# Autodesk Inventor assembly: BatteryPack
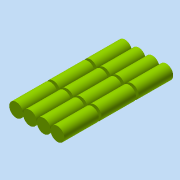
[picture p0: Inventor's stored thumbnail of the model, 180x180]
Saved by Autodesk Inventor 2015 (Build 190159000, 159)
## iProperties
Created: 2015-12-28
Part Number: BatteryPack
Document SubType Name: Assembly
Designer: Raphael
Author: Raphael
## Documents named in this file (2)
- \\psf\Home\Documents\electric-skateboard\CAD\BatteryPack.iam
- \\psf\Home\Documents\electric-skateboard\CAD\26650.ipt
## Components (12 placed, 1 different names)
1. 26650:1 — Mate:1, Mate:9, Flush:3, Tangent:2, Tangent:4
2. 26650:2 — Mate:1, Mate:2, Mate:9, Mate:10
3. 26650:3 — Mate:2, Mate:10
4. 26650:4 — Mate:3, Mate:11, Flush:2, Flush:3, Tangent:1, Tangent:2, Tangent:5
5. 26650:5 — Mate:3, Mate:4, Mate:11, Mate:12
6. 26650:6 — Mate:4, Mate:12
7. 26650:7 — Mate:5, Mate:13, Flush:1, Flush:2, Tangent:1, Tangent:3, Tangent:6
8. 26650:8 — Mate:5, Mate:6, Mate:13, Mate:14
9. 26650:9 — Mate:6, Mate:14
10. 26650:10 — Mate:7, Mate:15, Flush:1, Tangent:3, Tangent:7
11. 26650:11 — Mate:7, Mate:8, Mate:15, Mate:16
12. 26650:12 — Mate:8, Mate:16
## Relationships (26: Mate 16, Tangent 7, Flush 3)
- Mate:1 (5 mm): 26650:1 ↔ 26650:2
- Mate:2 (5 mm): 26650:2 ↔ 26650:3
- Mate:3 (5 mm): 26650:4 ↔ 26650:5
- Mate:4 (5 mm): 26650:5 ↔ 26650:6
- Mate:5 (5 mm): 26650:7 ↔ 26650:8
- Mate:6 (5 mm): 26650:8 ↔ 26650:9
- Mate:7 (5 mm): 26650:10 ↔ 26650:11
- Mate:8 (5 mm): 26650:11 ↔ 26650:12
- Mate:9: 26650:1 ↔ 26650:2
- Mate:10: 26650:2 ↔ 26650:3
- Mate:11: 26650:4 ↔ 26650:5
- Mate:12: 26650:5 ↔ 26650:6
- Mate:13: 26650:7 ↔ 26650:8
- Mate:14: 26650:8 ↔ 26650:9
- Mate:15: 26650:10 ↔ 26650:11
- Mate:16: 26650:11 ↔ 26650:12
- Flush:1: 26650:7 ↔ 26650:10
- Flush:2: 26650:4 ↔ 26650:7
- Flush:3: 26650:1 ↔ 26650:4
- Tangent:1: 26650:4 ↔ 26650:7
- Tangent:2: 26650:1 ↔ 26650:4
- Tangent:3: 26650:7 ↔ 26650:10
- Tangent:4: 26650:1
- Tangent:5: 26650:4
- Tangent:6: 26650:7
- Tangent:7: 26650:10
